# Autodesk Inventor assembly: _Tooling_PCBPaste
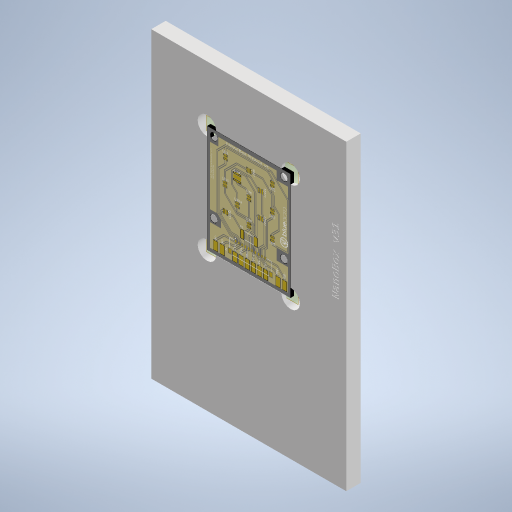
[picture p0: Inventor's stored thumbnail of the model, 512x512]
Saved by Autodesk Inventor 2023.2 (Build 272271030, 271C)
## iProperties
Created: 2023-03-08
Part Number: _Tooling_PCBPaste
Document SubType Name: Assembly
Designer: atrus
Author: atrus
## Documents named in this file (3)
- C:\Users\atrus\Dropbox\elec\Mechanical\NanoBoxArray\_Tooling_PCBPaste.iam
- C:\Users\atrus\Dropbox\elec\Mechanical\NanoBoxArray\PCB\nanobox_array_v31\nanobox_v31_upgrade_BOARD.ipt
- C:\Users\atrus\Dropbox\elec\Mechanical\NanoBoxArray\_Tooling_PCBPaste.ipt
## Components (2 placed, 2 different names)
1. nanobox_v31_upgrade_BOARD:1 — Flush:1, Flush:2
2. _Tooling_PCBPaste:1 — Flush:1, Flush:2
## Relationships (2: Flush 2)
- Flush:1: nanobox_v31_upgrade_BOARD:1 ↔ _Tooling_PCBPaste:1
- Flush:2: nanobox_v31_upgrade_BOARD:1 ↔ _Tooling_PCBPaste:1
